# Autodesk Inventor assembly: MyPart_V0_cam_layout
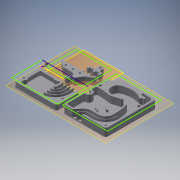
[picture p0: Inventor's stored thumbnail of the model, 180x180]
Saved by Autodesk Inventor 2016 (Build 200138000, 138)
## iProperties
Created: 2016-08-09
Part Number: MyPart_V0_cam_layout
Document SubType Name: Assembly
Designer: rawrdong
Author: rawrdong
## Documents named in this file (4)
- C:\Users\rawrdong\Box Sync\0_GradSchoolResearch\00_projects\0_AirParticleCounter\NEW_SHIT\MECH_E\MyPart_V0_cam_layout.iam
- C:\Users\rawrdong\Box Sync\0_GradSchoolResearch\00_projects\0_AirParticleCounter\NEW_SHIT\MECH_E\bottom_channel.ipt
- C:\Users\rawrdong\Box Sync\0_GradSchoolResearch\00_projects\0_AirParticleCounter\NEW_SHIT\MECH_E\top_channel.ipt
- C:\Users\rawrdong\Box Sync\0_GradSchoolResearch\00_projects\0_AirParticleCounter\NEW_SHIT\MECH_E\laser_holder.ipt
## Components (3 placed, 3 different names)
1. bottom_channel:1 — Mate:2, Mate:4
2. top_channel:1 — Mate:1
3. laser_holder:1 — Mate:3, Mate:4, Mate:5, Angle:1, Mate:6, Angle:2
## Relationships (8: Mate 6, Angle 2)
- Mate:1: top_channel:1
- Mate:2: bottom_channel:1
- Mate:3: laser_holder:1
- Mate:4 (10 mm): bottom_channel:1 ↔ laser_holder:1
- Mate:5: laser_holder:1
- Angle:1 (0 deg): laser_holder:1
- Mate:6: laser_holder:1
- Angle:2 (0 deg): laser_holder:1
